# Autodesk Inventor assembly: Aircraft Preliminary Design and W+B
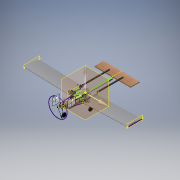
[picture p0: Inventor's stored thumbnail of the model, 180x180]
Saved by Autodesk Inventor 2018 (Build 220112000, 112)
## iProperties
Created: 2018-07-21
Part Number: Aircraft Preliminary Design and W+B
Document SubType Name: Assembly
Designer: Michael Gunderman
Mass: 3069.82 g
Surface Area: 15344.9 cm^2
Volume: 13743.9 cm^3
Density: 0.223358 g/cm^3
Author: Michael Gunderman
## Documents named in this file (12)
- C:\Users\Michael Gunderman\Documents\Special Projects\Echo 1\Echo-1-master\Echo 1\CAD work\Preliminary Shapes\Aircraft Preliminary Design and W+B.iam
- C:\Users\Michael Gunderman\Documents\Special Projects\Echo 1\Echo-1-master\Echo 1\CAD work\Systems\Electrical\Motor Turnigy G60 500kv.ipt
- C:\Users\Michael Gunderman\Documents\Special Projects\Echo 1\Echo-1-master\Echo 1\CAD work\Preliminary Shapes\Generic Wing 1.ipt
- C:\Users\Michael Gunderman\Documents\Special Projects\Echo 1\Echo-1-master\Echo 1\CAD work\Preliminary Shapes\Generic Tail 1.ipt
- C:\Users\Michael Gunderman\Documents\Special Projects\Echo 1\Echo-1-master\Echo 1\CAD work\Structures\500mm tube.ipt
- C:\Users\Michael Gunderman\Documents\Special Projects\Echo 1\Echo-1-master\Echo 1\CAD work\Systems\Electrical\Flight Battery 5000 mah 5S.ipt
- C:\Users\Michael Gunderman\Documents\Special Projects\Echo 1\Echo-1-master\Echo 1\CAD work\Preliminary Shapes\Main Landing Gear.ipt
- C:\Users\Michael Gunderman\Documents\Special Projects\Echo 1\Echo-1-master\Echo 1\CAD work\Systems\Landing Gear\Nose Gear Assembly.iam
- C:\Users\Michael Gunderman\Documents\Special Projects\Echo 1\Echo-1-master\Echo 1\CAD work\Systems\Payload\Bravo 1 Mockup.ipt
- C:\Users\Michael Gunderman\Documents\Special Projects\Echo 1\Echo-1-master\Echo 1\CAD work\Structures\All Structures Assembly.iam
- C:\Users\Michael Gunderman\Documents\Special Projects\Echo 1\Echo-1-master\Echo 1\CAD work\Structures\500mm tube_MIR1.ipt
- C:\Users\Michael Gunderman\Documents\Special Projects\Echo 1\Echo-1-master\Echo 1\CAD work\Preliminary Shapes\Generic Wing 1_MIR4.ipt
## Components (12 placed, 11 different names)
1. Motor Turnigy G60 500kv:1 — Mate:4, Mate:6
2. Generic Wing 1:1 — Mate:1
3. Generic Tail 1:1 — Mate:2
4. 500mm tube:1
5. Flight Battery 5000 mah 5S:1
6. Main Landing Gear:1
7. Main Landing Gear:2
8. Nose Gear Assembly:1 [sub-assembly]
9. Bravo 1 Mockup:1
10. All Structures Assembly:1 [sub-assembly] — Flush:2, Mate:5, Mate:6
11. 500mm tube_MIR1:1
12. Generic Wing 1_MIR4:1 — Mate:7
## Relationships (8: Mate 6, Flush 2)
- Flush:1 (143 mm)
- Mate:1: Generic Wing 1:1
- Mate:2: Generic Tail 1:1
- Mate:4: Motor Turnigy G60 500kv:1
- Flush:2: All Structures Assembly:1
- Mate:5: All Structures Assembly:1
- Mate:6: Motor Turnigy G60 500kv:1 ↔ All Structures Assembly:1
- Mate:7: Generic Wing 1_MIR4:1
